# Autodesk Inventor assembly: FullGripper
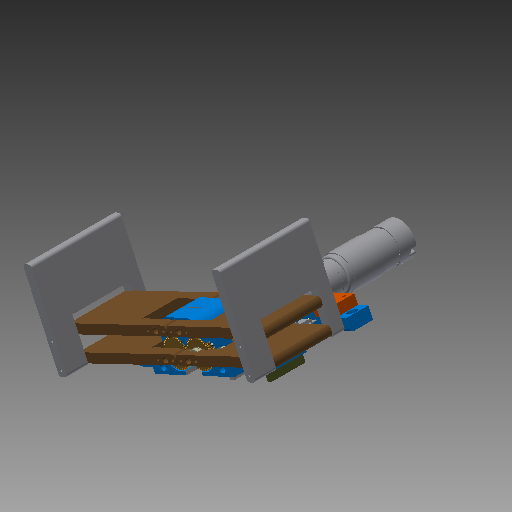
[picture p0: Inventor's stored thumbnail of the model, 512x512]
Saved by Autodesk Inventor 2019 (Build 230136000, 136)
## iProperties
Created: 2019-10-02
Part Number: FullGripper
Document SubType Name: Assembly
Designer: james
Author: james
## Documents named in this file (16)
- F:\JimsDesign\Jims2020FTC\FullGripper.iam
- F:\JimsDesign\Library\McMaster\57155K323_STAINLESS STEEL BALL BEARING.ipt
- F:\JimsDesign\Jims2020FTC\GripperAxle.ipt
- F:\JimsDesign\Library\ServoCity\625259.ipt
- F:\JimsDesign\Jims2020FTC\GripperGear.ipt
- F:\JimsDesign\Jims2020FTC\GripperArm.ipt
- F:\JimsDesign\Jims2020FTC\GripperPlate.ipt
- F:\JimsDesign\Jims2020FTC\GripperSidePlate.iam
- F:\JimsDesign\Library\McMaster\SocketScrews\91251A148_BLACK-OXIDE ALLOY STEEL SOCKET HEAD CAP SCREW.ipt
- F:\JimsDesign\Jims2020FTC\cLIMPpLATE.ipt
- F:\JimsDesign\Library\McMaster\7779K230_MINIATURE SNAP-ACTING SWITCH.ipt
- F:\JimsDesign\Jims2020FTC\GripperM otorBlock.ipt
- F:\JimsDesign\Library\ServoCity\5202-0002-0071 part.ipt
- F:\JimsDesign\Jims2020FTC\tOPgRIPPERcLAMP.ipt
- F:\JimsDesign\Jims2020FTC\FullGripperBlock.iam
- F:\JimsDesign\Jims2020FTC\TestPeg.ipt
## Components (28 placed, 15 different names)
1. 57155K323_STAINLESS STEEL BALL BEARING:1
2. 57155K323_STAINLESS STEEL BALL BEARING:2 — Mate:112
3. 57155K323_STAINLESS STEEL BALL BEARING:3 — Mate:114
4. 57155K323_STAINLESS STEEL BALL BEARING:4 — Mate:108
5. GripperAxle:1 — Mate:69, Mate:111, Mate:112, Mate:125, Mate:126
6. GripperAxle:2 — Mate:115, Mate:116, Mate:119, Mate:135
7. 625259:1 — Mate:69
8. GripperGear:1 — Mate:125, Flush:6
9. GripperGear:2 — Mate:116, Flush:2, Mate:120
10. GripperGear:3 — Mate:126, Flush:4, Mate:129, Mate:130, Mate:131
11. GripperGear:4 — Mate:115, Flush:5
12. GripperSidePlate:1 [sub-assembly] — Mate:139, Mate:140, Mate:141
13. GripperPlate:1 — Mate:152, Mate:153, Mate:154
14. GripperPlate:2 — Mate:149, Mate:150, Mate:151
15. 91251A148_BLACK-OXIDE ALLOY STEEL SOCKET HEAD CAP SCREW:1 — Mate:145, Mate:146
16. 91251A148_BLACK-OXIDE ALLOY STEEL SOCKET HEAD CAP SCREW:2 — Mate:147, Mate:148
17. cLIMPpLATE:1 — Mate:142, Mate:143, Mate:144, Mate:145, Mate:146, Mate:147, Mate:148
18. 7779K230_MINIATURE SNAP-ACTING SWITCH:1
19. GripperM otorBlock:1 — Mate:96, Mate:97, Mate:98, Mate:99, Mate:100, Mate:101, Mate:136, Mate:137, Mate:138, Mate:155, Mate:156, Flush:7
20. 5202-0002-0071 part:1 — Mate:155
21. tOPgRIPPERcLAMP:1 — Mate:99, Mate:100, Mate:101
22. tOPgRIPPERcLAMP:2 — Mate:96, Mate:97, Mate:98
23. FullGripperBlock:1 [sub-assembly] — Mate:108, Mate:111, Mate:114, Flush:2, Mate:117, Mate:118, Mate:121, Flush:4, Mate:127, Mate:128, Mate:135, Mate:136, Mate:137, Mate:138, Mate:139, Mate:140, Mate:141, Flush:5, Flush:6, Mate:142, Mate:143, Mate:144
24. GripperArm:1 — Mate:117, Mate:118, Mate:152, Mate:154
25. GripperArm:2 — Mate:119, Mate:120, Mate:121, Mate:153
26. GripperArm:3 — Mate:127, Mate:128, Mate:149, Mate:151
27. GripperArm:4 — Mate:129, Mate:130, Mate:131, Mate:150
28. TestPeg:1 — Mate:156, Flush:7
## Relationships (52: Mate 47, Flush 5)
- Mate:69: GripperAxle:1 ↔ 625259:1
- Mate:96: GripperM otorBlock:1 ↔ tOPgRIPPERcLAMP:2
- Mate:97: GripperM otorBlock:1 ↔ tOPgRIPPERcLAMP:2
- Mate:98: GripperM otorBlock:1 ↔ tOPgRIPPERcLAMP:2
- Mate:99: GripperM otorBlock:1 ↔ tOPgRIPPERcLAMP:1
- Mate:100: GripperM otorBlock:1 ↔ tOPgRIPPERcLAMP:1
- Mate:101: GripperM otorBlock:1 ↔ tOPgRIPPERcLAMP:1
- Mate:108: 57155K323_STAINLESS STEEL BALL BEARING:4 ↔ FullGripperBlock:1
- Mate:111: GripperAxle:1 ↔ FullGripperBlock:1
- Mate:112: 57155K323_STAINLESS STEEL BALL BEARING:2 ↔ GripperAxle:1
- Mate:114: 57155K323_STAINLESS STEEL BALL BEARING:3 ↔ FullGripperBlock:1
- Mate:115: GripperAxle:2 ↔ GripperGear:4
- Mate:116: GripperAxle:2 ↔ GripperGear:2
- Flush:2: GripperGear:2 ↔ FullGripperBlock:1
- Mate:117: FullGripperBlock:1 ↔ GripperArm:1
- Mate:118: FullGripperBlock:1 ↔ GripperArm:1
- Mate:119: GripperAxle:2 ↔ GripperArm:2
- Mate:120: GripperGear:2 ↔ GripperArm:2
- Mate:121: FullGripperBlock:1 ↔ GripperArm:2
- Mate:125: GripperAxle:1 ↔ GripperGear:1
- Mate:126: GripperAxle:1 ↔ GripperGear:3
- Flush:4: GripperGear:3 ↔ FullGripperBlock:1
- Mate:127: FullGripperBlock:1 ↔ GripperArm:3
- Mate:128: FullGripperBlock:1 ↔ GripperArm:3
- Mate:129: GripperGear:3 ↔ GripperArm:4
- Mate:130: GripperGear:3 ↔ GripperArm:4
- Mate:131: GripperGear:3 ↔ GripperArm:4
- Mate:135: GripperAxle:2 ↔ FullGripperBlock:1
- Mate:136: GripperM otorBlock:1 ↔ FullGripperBlock:1
- Mate:137: GripperM otorBlock:1 ↔ FullGripperBlock:1
- Mate:138: GripperM otorBlock:1 ↔ FullGripperBlock:1
- Mate:139: GripperSidePlate:1 ↔ FullGripperBlock:1
- Mate:140: GripperSidePlate:1 ↔ FullGripperBlock:1
- Mate:141: GripperSidePlate:1 ↔ FullGripperBlock:1
- Flush:5: GripperGear:4 ↔ FullGripperBlock:1
- Flush:6: GripperGear:1 ↔ FullGripperBlock:1
- Mate:142: cLIMPpLATE:1 ↔ FullGripperBlock:1
- Mate:143: cLIMPpLATE:1 ↔ FullGripperBlock:1
- Mate:144: cLIMPpLATE:1 ↔ FullGripperBlock:1
- Mate:145: 91251A148_BLACK-OXIDE ALLOY STEEL SOCKET HEAD CAP SCREW:1 ↔ cLIMPpLATE:1
- Mate:146: 91251A148_BLACK-OXIDE ALLOY STEEL SOCKET HEAD CAP SCREW:1 ↔ cLIMPpLATE:1
- Mate:147: 91251A148_BLACK-OXIDE ALLOY STEEL SOCKET HEAD CAP SCREW:2 ↔ cLIMPpLATE:1
- Mate:148: 91251A148_BLACK-OXIDE ALLOY STEEL SOCKET HEAD CAP SCREW:2 ↔ cLIMPpLATE:1
- Mate:149: GripperPlate:2 ↔ GripperArm:3
- Mate:150: GripperPlate:2 ↔ GripperArm:4
- Mate:151: GripperPlate:2 ↔ GripperArm:3
- Mate:152: GripperPlate:1 ↔ GripperArm:1
- Mate:153: GripperPlate:1 ↔ GripperArm:2
- Mate:154: GripperPlate:1 ↔ GripperArm:1
- Mate:155: GripperM otorBlock:1 ↔ 5202-0002-0071 part:1
- Mate:156: GripperM otorBlock:1 ↔ TestPeg:1
- Flush:7: GripperM otorBlock:1 ↔ TestPeg:1
